# Autodesk Inventor assembly: main room with double door
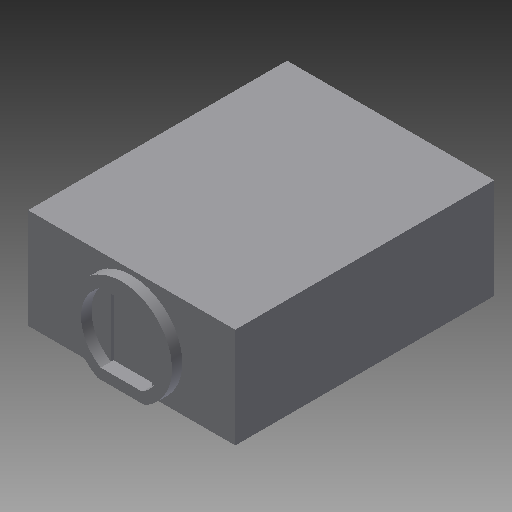
[picture p0: Inventor's stored thumbnail of the model, 512x512]
Saved by Autodesk Inventor 2017 (Build 210142000, 142)
## iProperties
Created: 2018-03-03
Part Number: main room with double door
Document SubType Name: Assembly
Designer: Braxton
Author: Braxton
## Documents named in this file (3)
- D:\School\Game develpment\geoscape\done\rooms\assembly\main room with double door.iam
- D:\School\Game develpment\geoscape\done\rooms\main room.ipt
- D:\School\Game develpment\geoscape\done\doors\double door.ipt
## Components (2 placed, 2 different names)
1. main room:1 — Mate:1, Mate:2, Mate:3
2. double door:1 — Mate:1, Mate:2, Mate:3
## Relationships (3: Mate 3)
- Mate:1: main room:1 ↔ double door:1
- Mate:2: main room:1 ↔ double door:1
- Mate:3: main room:1 ↔ double door:1
